# Autodesk Inventor assembly: Assembly
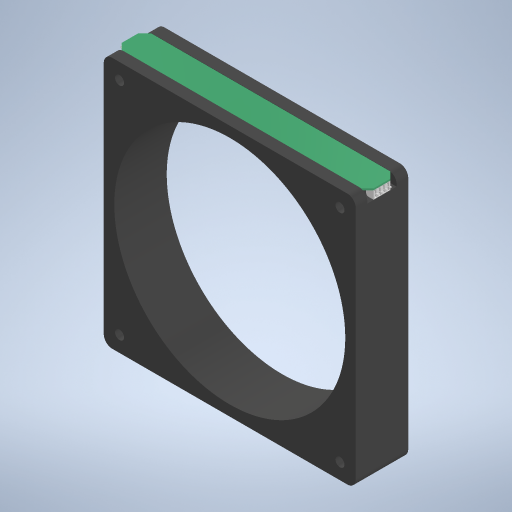
[picture p0: Inventor's stored thumbnail of the model, 512x512]
Saved by Autodesk Inventor 2023.1 (Build 271208000, 208)
## iProperties
Created: 2023-11-19
Part Number: Assembly
Document SubType Name: Assembly
Designer: Vinicius
Author: Vinicius
## iProperties of the stored document 476150001.ipt
Created: 2015-11-23
Part Number: 476150001
Material: Generic
Document SubType Name: Modeling
Designer: Vinicius
Appearance: Default
Sending System: PRO/ENGINEER BY PARAMETRIC TECHNOLOGY CORPORATION, 2011490
Preprocessor: PRO/ENGINEER BY PARAMETRIC TECHNOLOGY CORPORATION, 2011490
Title: 476150001
Author: gga
Revision Number: 1LAST_VERSION
## Documents named in this file (6)
- D:\Git\WirelessCommunicationCoolingFans\Mechanical\Assembly.iam
- FanAssembly.iam
- D:\Git\WirelessCommunicationCoolingFans\Mechanical\Body.ipt
- **D:\Git\WirelessCommunicationCoolingFans\Mechanical\Assembly.iam*LocalDocs*xAaaaamcaAaaaaaaaAaaaao2xRe*476150001.ipt
- D:\Git\WirelessCommunicationCoolingFans\Mechanical\PCB.ipt
- D:\Git\WirelessCommunicationCoolingFans\Mechanical\476150001.stp
## Components (4 placed, 3 different names)
1. Body:1 — Flush:1, Flush:2, Flush:5, Flush:6, Mate:1, Mate:2
2. 476150001:1 — Flush:1, Flush:3, Flush:4, Flush:5, Flush:6, Flush:7
3. 476150001:2 — Flush:2, Flush:3, Flush:4
4. PCB:1 — Mate:1, Mate:2, Flush:7
## Relationships (9: Flush 7, Mate 2)
- Flush:1: Body:1 ↔ 476150001:1
- Flush:2: Body:1 ↔ 476150001:2
- Flush:3: 476150001:1 ↔ 476150001:2
- Flush:4: 476150001:1 ↔ 476150001:2
- Flush:5: Body:1 ↔ 476150001:1
- Flush:6: Body:1 ↔ 476150001:1
- Mate:1: Body:1 ↔ PCB:1
- Mate:2: Body:1 ↔ PCB:1
- Flush:7: 476150001:1 ↔ PCB:1
